# Autodesk Inventor assembly: placa_galbena_composita
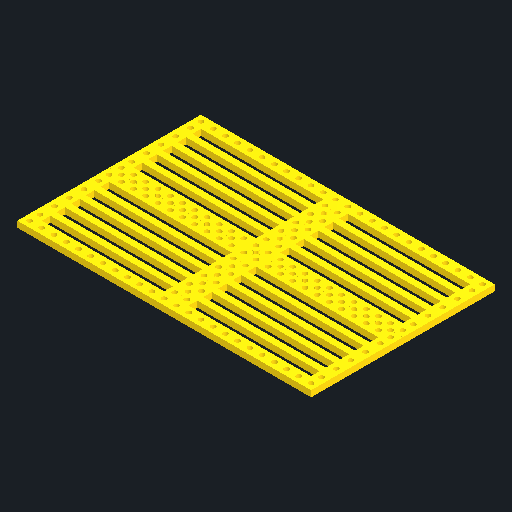
[picture p0: Inventor's stored thumbnail of the model, 512x512]
Saved by Autodesk Inventor 2026.1 (Build 301233000, 233)
## iProperties
Created: 2025-09-17
Part Number: placa_galbena_composita
Document SubType Name: Assembly
Designer: emanuel
Author: emanuel
## Documents named in this file (2)
- C:\Users\emanuel\UnFolder\SpiderRobo\3D_model\placa_galbena_composita.iam
- C:\Users\emanuel\UnFolder\SpiderRobo\3D_model\placa_galbena.ipt
## Components (4 placed, 1 different names)
1. placa_galbena:1 — Mate:2, Flush:3, Flush:4, Mate:3, Flush:5, Flush:6
2. placa_galbena:2 — Mate:1, Flush:1, Flush:2
3. placa_galbena:3 — Mate:1, Flush:1, Flush:2, Mate:3, Flush:5, Flush:6
4. placa_galbena:4 — Mate:2, Flush:3, Flush:4
## Relationships (9: Flush 6, Mate 3)
- Mate:1: placa_galbena:2 ↔ placa_galbena:3
- Flush:1: placa_galbena:2 ↔ placa_galbena:3
- Flush:2: placa_galbena:2 ↔ placa_galbena:3
- Mate:2: placa_galbena:1 ↔ placa_galbena:4
- Flush:3: placa_galbena:1 ↔ placa_galbena:4
- Flush:4: placa_galbena:1 ↔ placa_galbena:4
- Mate:3: placa_galbena:1 ↔ placa_galbena:3
- Flush:5: placa_galbena:1 ↔ placa_galbena:3
- Flush:6: placa_galbena:1 ↔ placa_galbena:3
